# Autodesk Inventor assembly: link_arm1_2
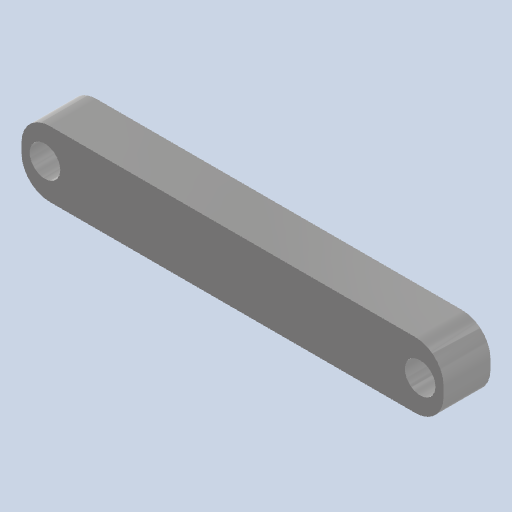
[picture p0: Inventor's stored thumbnail of the model, 512x512]
Saved by Autodesk Inventor 2025 (Build 290162000, 162)
## iProperties
Created: 2025-09-16
Part Number: link_arm1_2
Document SubType Name: Assembly
Designer: sooo1
Author: sooo1
## Documents named in this file (2)
- C:\Users\sooo1\Documents\Inventor\MOBITOUCH\final\stroke_module_1\link_arm1_2.iam
- C:\Users\sooo1\Documents\Inventor\MOBITOUCH\final\stroke_module_1\link_arm_1_2.ipt
## Components (1 placed, 1 different names)
1. link_arm_1_2:1 — フラッシュ:1, フラッシュ:2, フラッシュ:3
## Relationships (3: Flush 3)
- フラッシュ:1 [Flush]: link_arm_1_2:1
- フラッシュ:2 [Flush]: link_arm_1_2:1
- フラッシュ:3 [Flush]: link_arm_1_2:1
